# Autodesk Inventor assembly: CuboidSecurityBoxOpenedLayer
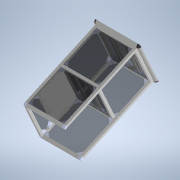
[picture p0: Inventor's stored thumbnail of the model, 180x180]
Saved by Autodesk Inventor 2021.1 (Build 251245010, 245A)
## iProperties
Created: 2020-11-09
Part Number: CuboidSecurityBoxOpenedLayer
Document SubType Name: Assembly
Designer: gisen
Author: gisen
## Documents named in this file (3)
- C:\Users\gisen\GitProjects\CAD-Data\CuboidAccessories\SecurityBox\CuboidSecurityBoxOpenedLayer.iam
- C:\Users\gisen\GitProjects\CAD-Data\CuboidAccessories\SecurityBox\Assemblies\CuboidSecurityBoxBasis.iam
- C:\Users\gisen\GitProjects\CAD-Data\CuboidAccessories\SecurityBox\Assemblies\AdditionalLayerAssembly.iam
## Components (2 placed, 2 different names)
1. CuboidSecurityBoxBasis:1 [sub-assembly] — フラッシュ:1, メイト:1, フラッシュ:2
2. AdditionalLayerAssembly:1 [sub-assembly] — フラッシュ:1, メイト:1, フラッシュ:2
## Relationships (3: Flush 2, Mate 1)
- フラッシュ:1 [Flush] (20 mm): CuboidSecurityBoxBasis:1 ↔ AdditionalLayerAssembly:1
- メイト:1 [Mate]: CuboidSecurityBoxBasis:1 ↔ AdditionalLayerAssembly:1
- フラッシュ:2 [Flush]: CuboidSecurityBoxBasis:1 ↔ AdditionalLayerAssembly:1
